(part 1 of 2)
# Autodesk Inventor assembly: gasienica_zlozenie
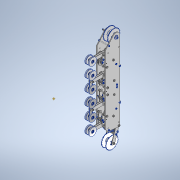
[picture p0: Inventor's stored thumbnail of the model, 180x180]
Saved by Autodesk Inventor 2020.3 (Build 243373000, 373)
## iProperties
Created: 2021-10-24
Part Number: gasienica_zlozenie
Document SubType Name: Assembly
Designer: patry
Author: patry
## Documents named in this file (46)
- C:\Users\patry\Desktop\Semestr 7\Inzynierka\Projekt inventor\Ariadna_inzynierka\Workspaces\Obszar roboczy\Obszar roboczy\Naped\Zawieszenie_v3\gasienica_zlozenie.iam
- C:\Users\patry\Desktop\Semestr 7\Inzynierka\Projekt inventor\Ariadna_inzynierka\Workspaces\Obszar roboczy\Obszar roboczy\Naped\Kola\kolo_przednie.iam
- C:\Users\patry\Desktop\Semestr 7\Inzynierka\Projekt inventor\Ariadna_inzynierka\Workspaces\Obszar roboczy\Obszar roboczy\Naped\Sruby\M5x65.ipt
- C:\Users\patry\Desktop\Semestr 7\Inzynierka\Projekt inventor\Ariadna_inzynierka\Workspaces\Obszar roboczy\Obszar roboczy\Naped\Sruby\M5_nut_5mm.ipt
- C:\Users\patry\Desktop\Semestr 7\Inzynierka\Projekt inventor\Ariadna_inzynierka\Workspaces\Obszar roboczy\Obszar roboczy\Naped\Sruby\dystans_miedzy_plytami.ipt
- C:\Users\patry\Desktop\Semestr 7\Inzynierka\Projekt inventor\Ariadna_inzynierka\Workspaces\Obszar roboczy\Obszar roboczy\Naped\Zawieszenie_v3\tuleja_TUF106040.ipt
- C:\Users\patry\Desktop\Semestr 7\Inzynierka\Projekt inventor\Ariadna_inzynierka\Workspaces\Obszar roboczy\Obszar roboczy\Naped\Sruby\M6_nut_5mm.ipt
- C:\Users\patry\Desktop\Semestr 7\Inzynierka\Projekt inventor\Ariadna_inzynierka\Workspaces\Obszar roboczy\Obszar roboczy\Naped\Amortyzator\Korpus.ipt
- C:\Users\patry\Desktop\Semestr 7\Inzynierka\Projekt inventor\Ariadna_inzynierka\Workspaces\Obszar roboczy\Obszar roboczy\Naped\Amortyzator\Tlok.ipt
- C:\Users\patry\Desktop\Semestr 7\Inzynierka\Projekt inventor\Ariadna_inzynierka\Workspaces\Obszar roboczy\Obszar roboczy\Naped\Amortyzator\Nakretka.ipt
- C:\Users\patry\Desktop\Semestr 7\Inzynierka\Projekt inventor\Ariadna_inzynierka\Workspaces\Obszar roboczy\Obszar roboczy\Naped\Sruby\M8_nut_6.5mm_MIR1.ipt
- C:\Users\patry\Desktop\Semestr 7\Inzynierka\Projekt inventor\Ariadna_inzynierka\Workspaces\Obszar roboczy\Obszar roboczy\Naped\Sruby\M8x80_threaded_MIR1.ipt
- C:\Users\patry\Desktop\Semestr 7\Inzynierka\Projekt inventor\Ariadna_inzynierka\Workspaces\Obszar roboczy\Obszar roboczy\Naped\Sruby\M8_pad_MIR1.ipt
- C:\Users\patry\Desktop\Semestr 7\Inzynierka\Projekt inventor\Ariadna_inzynierka\Workspaces\Obszar roboczy\Obszar roboczy\Naped\Lozyska\608ZZ-8mm\bearings-608zz-80018-1.snapshot.1\608zz_MIR1.ipt
- C:\Users\patry\Desktop\Semestr 7\Inzynierka\Projekt inventor\Ariadna_inzynierka\Workspaces\Obszar roboczy\Obszar roboczy\Naped\Kola\kolo_napedowe.iam
- C:\Users\patry\Desktop\Semestr 7\Inzynierka\Projekt inventor\Ariadna_inzynierka\Workspaces\Obszar roboczy\Obszar roboczy\Naped\Sruby\M5_70_shaft.ipt
- C:\Users\patry\Desktop\Semestr 7\Inzynierka\Projekt inventor\Ariadna_inzynierka\Workspaces\Obszar roboczy\Obszar roboczy\Naped\Sruby\M3_16_shaft.ipt
- C:\Users\patry\Desktop\Semestr 7\Inzynierka\Projekt inventor\Ariadna_inzynierka\Workspaces\Obszar roboczy\Obszar roboczy\Naped\Sruby\M3_nut_2,5mm.ipt
- C:\Users\patry\Desktop\Semestr 7\Inzynierka\Projekt inventor\Ariadna_inzynierka\Workspaces\Obszar roboczy\Obszar roboczy\Naped\Zawieszenie_v3\wspornik_amortyzatora.ipt
- C:\Users\patry\Desktop\Semestr 7\Inzynierka\Projekt inventor\Ariadna_inzynierka\Workspaces\Obszar roboczy\Obszar roboczy\Naped\Sruby\M6_70_shaft.ipt
- C:\Users\patry\Desktop\Semestr 7\Inzynierka\Projekt inventor\Ariadna_inzynierka\Workspaces\Obszar roboczy\Obszar roboczy\Naped\Sruby\tuleja_M5_M9_20.ipt
- C:\Users\patry\Desktop\Semestr 7\Inzynierka\Projekt inventor\Ariadna_inzynierka\Workspaces\Obszar roboczy\Obszar roboczy\Naped\Sruby\tuleja_M5_M9_25.ipt
- C:\Users\patry\Desktop\Semestr 7\Inzynierka\Projekt inventor\Ariadna_inzynierka\Workspaces\Obszar roboczy\Obszar roboczy\Naped\Kola\holder_wheel_pair.iam
- C:\Users\patry\Desktop\Semestr 7\Inzynierka\Projekt inventor\Ariadna_inzynierka\Workspaces\Obszar roboczy\Obszar roboczy\Naped\Zawieszenie_v3\ramie_napinacza.ipt
- C:\Users\patry\Desktop\Semestr 7\Inzynierka\Projekt inventor\Ariadna_inzynierka\Workspaces\Obszar roboczy\Obszar roboczy\Naped\Sruby\M5_60_shaft.ipt
- C:\Users\patry\Desktop\Semestr 7\Inzynierka\Projekt inventor\Ariadna_inzynierka\Workspaces\Obszar roboczy\Obszar roboczy\Naped\Sruby\tuleja_M5_M9_13.ipt
- C:\Users\patry\Desktop\Semestr 7\Inzynierka\Projekt inventor\Ariadna_inzynierka\Workspaces\Obszar roboczy\Obszar roboczy\Naped\Sruby\tuleja_M5_M9_18.ipt
- C:\Users\patry\Desktop\Semestr 7\Inzynierka\Projekt inventor\Ariadna_inzynierka\Workspaces\Obszar roboczy\Obszar roboczy\Naped\Sruby\tuleja_M6_M10_8.ipt
- C:\Users\patry\Desktop\Semestr 7\Inzynierka\Projekt inventor\Ariadna_inzynierka\Workspaces\Obszar roboczy\Obszar roboczy\Naped\Zawieszenie_v3\plyta_boczna.ipt
- C:\Users\patry\Desktop\Semestr 7\Inzynierka\Projekt inventor\Ariadna_inzynierka\Workspaces\Obszar roboczy\Obszar roboczy\Naped\Zawieszenie_v3\ramie_1_wahacza.ipt
- C:\Users\patry\Desktop\Semestr 7\Inzynierka\Projekt inventor\Ariadna_inzynierka\Workspaces\Obszar roboczy\Obszar roboczy\Naped\Zawieszenie_v3\ramie_2_wahacza.ipt
- C:\Users\patry\Desktop\Semestr 7\Inzynierka\Projekt inventor\Ariadna_inzynierka\Workspaces\Obszar roboczy\Obszar roboczy\Naped\Sruby\M6_40_shaft.ipt
- C:\Users\patry\Desktop\Semestr 7\Inzynierka\Projekt inventor\Ariadna_inzynierka\Workspaces\Obszar roboczy\Obszar roboczy\Naped\Sruby\tuleja_M6_M10_7.ipt
- C:\Users\patry\Desktop\Semestr 7\Inzynierka\Projekt inventor\Ariadna_inzynierka\Workspaces\Obszar roboczy\Obszar roboczy\Naped\Sruby\M6_1,25_pad.ipt
- C:\Users\patry\Desktop\Semestr 7\Inzynierka\Projekt inventor\Ariadna_inzynierka\Workspaces\Obszar roboczy\Obszar roboczy\Naped\Sruby\M5_40_shaft.ipt
- M5_shaft.ipt
- C:\Users\patry\Desktop\Semestr 7\Inzynierka\Projekt inventor\Ariadna_inzynierka\Workspaces\Obszar roboczy\Obszar roboczy\Naped\Sruby\tuleja_M5_M9_4,5.ipt
- C:\Users\patry\Desktop\Semestr 7\Inzynierka\Projekt inventor\Ariadna_inzynierka\Workspaces\Obszar roboczy\Obszar roboczy\Naped\Zawieszenie_v3\glowny_wahacz_zewn.ipt
- C:\Users\patry\Desktop\Semestr 7\Inzynierka\Projekt inventor\Ariadna_inzynierka\Workspaces\Obszar roboczy\Obszar roboczy\Naped\Zawieszenie_v3\independent_wheel_pair.iam
- C:\Users\patry\Desktop\Semestr 7\Inzynierka\Projekt inventor\Ariadna_inzynierka\Workspaces\Obszar roboczy\Obszar roboczy\Naped\Sruby\tuleja_M6_M10_6.ipt
- C:\Users\patry\Desktop\Semestr 7\Inzynierka\Projekt inventor\Ariadna_inzynierka\Workspaces\Obszar roboczy\Obszar roboczy\Naped\Sruby\tuleja_M5_M9_17.5.ipt
- C:\Users\patry\Desktop\Semestr 7\Inzynierka\Projekt inventor\Ariadna_inzynierka\Workspaces\Obszar roboczy\Obszar roboczy\Naped\Zawieszenie_v3\komplet_kol_V4.iam
- C:\Users\patry\Desktop\Semestr 7\Inzynierka\Projekt inventor\Ariadna_inzynierka\Workspaces\Obszar roboczy\Obszar roboczy\Naped\Sruby\M6_25_shaft.ipt
- C:\Users\patry\Desktop\Semestr 7\Inzynierka\Projekt inventor\Ariadna_inzynierka\Workspaces\Obszar roboczy\Obszar roboczy\Naped\Kola\single_wheel_dummie.iam
- C:\Users\patry\Desktop\Semestr 7\Inzynierka\Projekt inventor\Ariadna_inzynierka\Workspaces\Obszar roboczy\Obszar roboczy\Naped\Sruby\tuleja_M5_M10_15.ipt
- C:\Users\patry\Desktop\Semestr 7\Inzynierka\Projekt inventor\Ariadna_inzynierka\Workspaces\Obszar roboczy\Obszar roboczy\Naped\Sruby\tuleja_M6_M10_7,5.ipt
## Components (345 placed, 44 different names)
1. M5x65:3
2. M5_nut_5mm:3
3. dystans_miedzy_plytami:3
4. M8_nut_6.5mm_MIR1:1
5. M8x80_threaded_MIR1:1
6. M8_nut_6.5mm_MIR1:2
7. M8_nut_6.5mm_MIR1:3
8. M8_pad_MIR1:1
9. M8_pad_MIR1:2
10. M8_pad_MIR1:3
11. M8_pad_MIR1:4
12. 608zz_MIR1:1
13. 608zz_MIR1:2 — Zestawiające:1077, Równoległe:74
14. kolo_napedowe:1 [sub-assembly]
15. kolo_przednie:1 [sub-assembly]
16. ramie_napinacza:1 — Zestawiające:1807
17. Korpus:6 — Walcowe:6
18. Tlok:6 — Walcowe:6
19. Nakretka:6
20. M5_nut_5mm:34
21. M5_70_shaft:6 — Zestawiające:1080
22. M5_nut_5mm:35
23. M3_16_shaft:6
24. M3_nut_2,5mm:11
25. M3_nut_2,5mm:12
26. wspornik_amortyzatora:11 — Zestawiające:1086, Zestawiające:1087
27. wspornik_amortyzatora:12
28. M5_nut_5mm:36
29. M5_nut_5mm:37
30. M5_nut_5mm:38
31. M5_nut_5mm:39
32. tuleja_M5_M9_20:6
33. tuleja_M5_M9_25:6
34. ramie_napinacza:2 — Zestawiające:1804
35. M5_60_shaft:1 — Zestawiające:1086
36. M5_60_shaft:2 — Zestawiające:1087, Zestawiające:1796, Zestawiające:1797
37. tuleja_TUF106040:41 — Zestawiające:1085
38. tuleja_TUF106040:42
39. M6_70_shaft:11 — Zestawiające:1079, Zestawiające:1802, Zestawiające:1803, Zestawiające:1806
40. M6_nut_5mm:49
41. M6_nut_5mm:50
42. tuleja_M5_M9_13:1 — Zestawiające:1796
43. tuleja_M5_M9_18:1 — Zestawiające:1797
44. M6_70_shaft:12
45. M6_nut_5mm:51
46. M6_nut_5mm:52
47. tuleja_M6_M10_8:1
48. tuleja_M6_M10_8:2
49. holder_wheel_pair:4 [sub-assembly] — Zestawiające:1082, Zestawiające:1083
50. holder_wheel_pair:5 [sub-assembly] — Zestawiające:1081, Zestawiające:1084
51. plyta_boczna:1 — Zestawiające:1075, Zestawiające:1076, Zestawiające:1077, Zestawiające:1078, Równoległe:74, Kątowe:22, Zestawiające:1079, Zestawiające:1080, Zestawiające:1081, Zestawiające:1082, Zestawiające:1083, Zestawiające:1084, Zestawiające:1085, Zestawiające:1632, Zestawiające:1633, Kątowe:49
52. plyta_boczna:2 — Zestawiające:1075, Zestawiające:1076, Zestawiające:1078, Zestawiające:1222, Zestawiające:1224, Zestawiające:1225, Zestawiające:1226, Zestawiające:1636, Zestawiające:1637, Zestawiające:1638, Zestawiające:1639, Zestawiające:1640, Zestawiające:1641, Zestawiające:1777, Zestawiające:1778, Zestawiające:1779, Zestawiające:1780
53. ramie_1_wahacza:1
54. ramie_2_wahacza:1
55. tuleja_TUF106040:43
56. tuleja_TUF106040:44
57. tuleja_TUF106040:45
58. tuleja_TUF106040:46
59. tuleja_TUF106040:47
60. tuleja_TUF106040:48
61. ramie_2_wahacza:2
62. tuleja_TUF106040:49
63. tuleja_TUF106040:50
64. M6_nut_5mm:53
65. Korpus:7
66. Tlok:7
67. Nakretka:7
68. M5_nut_5mm:40
69. M5_70_shaft:7
70. ramie_1_wahacza:2 — Kątowe:27
71. M5_nut_5mm:41
72. M3_16_shaft:7
73. M3_nut_2,5mm:13
74. M3_nut_2,5mm:14
75. wspornik_amortyzatora:13
76. wspornik_amortyzatora:14
77. M6_40_shaft:1
78. M6_40_shaft:2
79. M6_nut_5mm:54
80. M6_nut_5mm:55
81. M6_nut_5mm:56
82. tuleja_M6_M10_7:1
83. tuleja_M6_M10_7:2
84. M6_1,25_pad:1
85. M6_1,25_pad:2
86. M6_1,25_pad:3
87. M6_1,25_pad:4
88. M6_1,25_pad:5
89. M6_1,25_pad:6
90. M6_1,25_pad:7
91. M6_1,25_pad:8
92. M6_70_shaft:13 — Zestawiające:1225
93. M6_70_shaft:14 — Zestawiające:1222
94. M6_nut_5mm:57
95. M6_nut_5mm:58 — Zestawiające:1224
96. M6_nut_5mm:59
97. M6_nut_5mm:60
98. M5_shaft:1
99. M5_shaft:2
100. M5_nut_5mm:42
101. M5_nut_5mm:43
102. M5_nut_5mm:44
103. M5_nut_5mm:45
104. tuleja_M5_M9_4,5:1
105. tuleja_M5_M9_4,5:2
106. tuleja_M5_M9_4,5:3
107. tuleja_M5_M9_4,5:4
108. glowny_wahacz_zewn:1 — Zestawiające:1223, Kątowe:27
109. glowny_wahacz_zewn:2
110. independent_wheel_pair:1 [sub-assembly]
111. tuleja_M6_M10_7:3 — Zestawiające:1223
112. tuleja_M6_M10_6:1
113. M6_nut_5mm:61
114. M6_nut_5mm:62
115. M6_nut_5mm:63
116. M6_nut_5mm:64
117. tuleja_M6_M10_6:2
118. tuleja_M6_M10_6:3
119. tuleja_M6_M10_6:4
120. M5_nut_5mm:46
121. M5_nut_5mm:47
122. tuleja_M5_M9_17.5:1
123. tuleja_M5_M9_17.5:2 — Zestawiające:1226
124. ramie_1_wahacza:3
125. ramie_2_wahacza:3
126. tuleja_TUF106040:51
127. tuleja_TUF106040:52
128. tuleja_TUF106040:53
129. tuleja_TUF106040:54
130. tuleja_TUF106040:55
131. tuleja_TUF106040:56
132. ramie_2_wahacza:4
133. tuleja_TUF106040:57
134. tuleja_TUF106040:58
135. M6_nut_5mm:65
136. Korpus:8
137. Tlok:8
138. Nakretka:8
139. M5_nut_5mm:48
140. M5_70_shaft:8
141. ramie_1_wahacza:4 — Kątowe:40
142. M5_nut_5mm:49
143. M3_16_shaft:8
144. M3_nut_2,5mm:15
145. M3_nut_2,5mm:16
146. wspornik_amortyzatora:15
147. wspornik_amortyzatora:16
148. M6_40_shaft:3
149. M6_40_shaft:4
150. M6_nut_5mm:66
151. M6_nut_5mm:67
152. M6_nut_5mm:68
153. tuleja_M6_M10_7:4
154. tuleja_M6_M10_7:5
155. M6_1,25_pad:9
156. M6_1,25_pad:10
157. M6_1,25_pad:11
158. M6_1,25_pad:12
159. M6_1,25_pad:13
160. M6_1,25_pad:14
161. M6_1,25_pad:15
162. M6_1,25_pad:16
163. M6_70_shaft:15 — Zestawiające:1636
164. M6_70_shaft:16 — Zestawiające:1632
165. M6_nut_5mm:69
166. M6_nut_5mm:70
167. M6_nut_5mm:71
168. M6_nut_5mm:72
169. M5_shaft:3
170. M5_shaft:4
171. M5_nut_5mm:50
172. M5_nut_5mm:51
173. M5_nut_5mm:52
174. M5_nut_5mm:53
175. tuleja_M5_M9_4,5:5
176. tuleja_M5_M9_4,5:6
177. tuleja_M5_M9_4,5:7
178. tuleja_M5_M9_4,5:8
179. glowny_wahacz_zewn:3 — Kątowe:40, Zestawiające:1793, Zestawiające:1794, Zestawiające:1795
180. glowny_wahacz_zewn:4 — Zestawiające:1793
181. tuleja_M6_M10_6:5
182. M6_nut_5mm:73
183. M6_nut_5mm:74
184. M6_nut_5mm:75 — Zestawiające:1633
185. M6_nut_5mm:76
186. tuleja_M6_M10_6:6
187. tuleja_M6_M10_6:7
188. tuleja_M6_M10_6:8
189. M5_nut_5mm:54
190. M5_nut_5mm:55
191. tuleja_M5_M9_17.5:3 — Zestawiające:1637
192. tuleja_M5_M9_17.5:4
193. ramie_1_wahacza:7 — Kątowe:41
194. ramie_2_wahacza:7
195. tuleja_TUF106040:67
196. tuleja_TUF106040:68
197. tuleja_TUF106040:69
198. tuleja_TUF106040:70
199. tuleja_TUF106040:71
200. tuleja_TUF106040:72
201. ramie_2_wahacza:8
202. tuleja_TUF106040:73
203. tuleja_TUF106040:74
204. M6_nut_5mm:89
205. Korpus:10
206. Tlok:10
207. Nakretka:10
208. M5_nut_5mm:64
209. M5_70_shaft:10
210. ramie_1_wahacza:8
211. M5_nut_5mm:65 — Zestawiające:1638
212. M3_16_shaft:10
213. M3_nut_2,5mm:19
214. M3_nut_2,5mm:20
215. wspornik_amortyzatora:19
216. wspornik_amortyzatora:20
217. M6_40_shaft:7
218. M6_40_shaft:8
219. M6_nut_5mm:90
220. M6_nut_5mm:91
221. M6_nut_5mm:92
222. tuleja_M6_M10_7:10
223. tuleja_M6_M10_7:11
224. M6_1,25_pad:25
225. M6_1,25_pad:26
226. M6_1,25_pad:27
227. M6_1,25_pad:28
228. M6_1,25_pad:29
229. M6_1,25_pad:30
230. M6_1,25_pad:31
231. M6_1,25_pad:32
232. M6_70_shaft:19 — Zestawiające:1640
233. M6_70_shaft:20 — Zestawiające:1639
234. M6_nut_5mm:93
235. M6_nut_5mm:94
236. M6_nut_5mm:95
237. M6_nut_5mm:96
238. M5_shaft:7
239. M5_shaft:8
240. M5_nut_5mm:66
241. M5_nut_5mm:67
242. M5_nut_5mm:68
243. M5_nut_5mm:69
244. tuleja_M5_M9_4,5:13
245. tuleja_M5_M9_4,5:14
246. tuleja_M5_M9_4,5:15
247. tuleja_M5_M9_4,5:16
248. glowny_wahacz_zewn:7 — Zestawiające:1784
249. glowny_wahacz_zewn:8 — Kątowe:41, Zestawiające:1781, Zestawiające:1782, Zestawiające:1789
250. tuleja_M6_M10_6:13
251. M6_nut_5mm:97
252. M6_nut_5mm:98
253. M6_nut_5mm:99
254. M6_nut_5mm:100
255. tuleja_M6_M10_6:14
256. tuleja_M6_M10_6:15
257. tuleja_M6_M10_6:16
258. M5_nut_5mm:70
259. M5_nut_5mm:71
260. tuleja_M5_M9_17.5:7 — Zestawiające:1641
261. tuleja_M5_M9_17.5:8
262. ramie_1_wahacza:9 — Kątowe:47
263. ramie_2_wahacza:9
264. tuleja_TUF106040:75
265. tuleja_TUF106040:76
266. tuleja_TUF106040:77
267. tuleja_TUF106040:78
268. tuleja_TUF106040:79
269. tuleja_TUF106040:80
270. ramie_2_wahacza:10
271. tuleja_TUF106040:81
272. tuleja_TUF106040:82
273. M6_nut_5mm:101
274. Korpus:11
275. Tlok:11
276. Nakretka:11
277. M5_nut_5mm:72
278. M5_70_shaft:11
279. ramie_1_wahacza:10
280. M5_nut_5mm:73
281. M3_16_shaft:11
282. M3_nut_2,5mm:21
283. M3_nut_2,5mm:22
284. wspornik_amortyzatora:21
285. wspornik_amortyzatora:22
286. M6_40_shaft:9
287. M6_40_shaft:10
288. M6_nut_5mm:102
289. M6_nut_5mm:103
290. M6_nut_5mm:104
291. tuleja_M6_M10_7:13
292. tuleja_M6_M10_7:14
293. M6_1,25_pad:33
294. M6_1,25_pad:34
295. M6_1,25_pad:35
296. M6_1,25_pad:36
297. M6_1,25_pad:37
298. M6_1,25_pad:38
299. M6_1,25_pad:39
300. M6_1,25_pad:40
301. M6_70_shaft:21 — Zestawiające:1779
302. M6_70_shaft:22 — Zestawiające:1778
303. M6_nut_5mm:105
304. M6_nut_5mm:106
305. M6_nut_5mm:107 — Zestawiające:1777
306. M6_nut_5mm:108
307. M5_shaft:9
308. M5_shaft:10
309. M5_nut_5mm:74
310. M5_nut_5mm:75
311. M5_nut_5mm:76
312. M5_nut_5mm:77
313. tuleja_M5_M9_4,5:17
314. tuleja_M5_M9_4,5:18
315. tuleja_M5_M9_4,5:19
316. tuleja_M5_M9_4,5:20
317. glowny_wahacz_zewn:9
318. glowny_wahacz_zewn:10 — Kątowe:47
319. independent_wheel_pair:5 [sub-assembly]
320. tuleja_M6_M10_7:15
321. tuleja_M6_M10_6:17
322. M6_nut_5mm:109
323. M6_nut_5mm:110
324. M6_nut_5mm:111
325. M6_nut_5mm:112
326. tuleja_M6_M10_6:18
327. tuleja_M6_M10_6:19
328. tuleja_M6_M10_6:20
329. M5_nut_5mm:78
330. M5_nut_5mm:79
331. tuleja_M5_M9_17.5:9
332. tuleja_M5_M9_17.5:10 — Zestawiające:1780
333. komplet_kol_V4:1 [sub-assembly] — Zestawiające:1781, Zestawiające:1782, Zestawiające:1784, Zestawiające:1788, Kątowe:48
334. M6_nut_5mm:115 — Zestawiające:1789
335. M6_25_shaft:2 — Zestawiające:1788
336. M6_nut_5mm:116
337. komplet_kol_V4:2 [sub-assembly] — Zestawiające:1795, Kątowe:48, Kątowe:49
338. M6_nut_5mm:117
339. M6_25_shaft:3 — Zestawiające:1794
340. M6_nut_5mm:118
341. single_wheel_dummie:1 [sub-assembly] — Zestawiające:1799
342. single_wheel_dummie:2 [sub-assembly] — Zestawiające:1800, Zestawiające:1801, Zestawiające:1802, Zestawiające:1805
343. tuleja_M5_M10_15:1 — Zestawiające:1799, Zestawiające:1800, Zestawiające:1801
344. tuleja_M6_M10_7,5:1 — Zestawiające:1803, Zestawiające:1804, Zestawiające:1805
345. tuleja_M6_M10_7,5:2 — Zestawiające:1806, Zestawiające:1807
## Relationships (742: Mate 664, Flush 49, Angle 24, CylindricalJoint 5)
- [Mate]: M5x65:3 ↔ M5_nut_5mm:3
- [Flush]: M5x65:3 ↔ M5_nut_5mm:3
- [Mate]: M5x65:3 ↔ dystans_miedzy_plytami:3
- [Mate] (5 mm): M5x65:3 ↔ dystans_miedzy_plytami:3
- [Mate]: M8_nut_6.5mm_MIR1:1 ↔ M8x80_threaded_MIR1:1
- [Mate]: M8x80_threaded_MIR1:1 ↔ M8_nut_6.5mm_MIR1:2
- [Mate]: M8x80_threaded_MIR1:1 ↔ M8_nut_6.5mm_MIR1:3
- [Mate]: M8_nut_6.5mm_MIR1:1 ↔ M8_pad_MIR1:1
- [Mate] (7 mm): M8x80_threaded_MIR1:1 ↔ M8_pad_MIR1:1
- [Mate]: M8x80_threaded_MIR1:1 ↔ M8_pad_MIR1:1
- [Mate]: M8_nut_6.5mm_MIR1:1 ↔ M8_pad_MIR1:2
- [Mate]: M8x80_threaded_MIR1:1 ↔ M8_pad_MIR1:2
- [Mate] (7 mm): M8_nut_6.5mm_MIR1:2 ↔ M8_pad_MIR1:3
- [Mate]: M8_nut_6.5mm_MIR1:3 ↔ M8_pad_MIR1:3
- [Mate]: M8x80_threaded_MIR1:1 ↔ M8_pad_MIR1:3
- [Mate]: M8_nut_6.5mm_MIR1:3 ↔ M8_pad_MIR1:4
- [Mate] (31 mm): M8_pad_MIR1:2 ↔ M8_pad_MIR1:4
- [Mate]: M8x80_threaded_MIR1:1 ↔ M8_pad_MIR1:4
- [Mate]: M8x80_threaded_MIR1:1 ↔ 608zz_MIR1:1
- [Mate]: M8_nut_6.5mm_MIR1:2 ↔ 608zz_MIR1:1
- [Mate]: M8x80_threaded_MIR1:1 ↔ 608zz_MIR1:2
- [Mate]: M8x80_threaded_MIR1:1 ↔ 608zz_MIR1:2
- [Mate]: M8x80_threaded_MIR1:1 ↔ kolo_napedowe:1
- [Mate]: M8_pad_MIR1:2 ↔ kolo_napedowe:1
- [Mate]: Korpus:6 ↔ Tlok:6
- [Angle] (0 deg): Korpus:6 ↔ Tlok:6
- [Mate]: Korpus:6 ↔ Nakretka:6
- [Mate] (5 mm): Korpus:6 ↔ Nakretka:6
- Walcowe:6 [CylindricalJoint]: Korpus:6 ↔ Tlok:6
- [Mate]: Korpus:6 ↔ M5_70_shaft:6
- [Flush] (-30 mm): Korpus:6 ↔ M5_70_shaft:6
- [Mate]: M5_nut_5mm:34 ↔ M5_70_shaft:6
- [Mate]: M5_70_shaft:6 ↔ M5_nut_5mm:35
- [Mate] (60 mm): M5_nut_5mm:34 ↔ M5_nut_5mm:35
- [Mate] (30 mm): Korpus:6 ↔ M5_nut_5mm:34
- [Mate]: wspornik_amortyzatora:11 ↔ wspornik_amortyzatora:12
- [Mate]: wspornik_amortyzatora:11 ↔ wspornik_amortyzatora:12
- [Mate] (5 mm): wspornik_amortyzatora:11 ↔ wspornik_amortyzatora:12
- [Mate]: M3_16_shaft:6 ↔ wspornik_amortyzatora:12
- [Flush] (-2.5 mm): M3_16_shaft:6 ↔ wspornik_amortyzatora:11
- [Mate]: M3_16_shaft:6 ↔ M3_nut_2,5mm:11
- [Mate]: M3_nut_2,5mm:11 ↔ wspornik_amortyzatora:11
- [Mate]: M3_16_shaft:6 ↔ M3_nut_2,5mm:12
- [Mate]: M3_nut_2,5mm:12 ↔ wspornik_amortyzatora:12
- [Mate]: Tlok:6 ↔ M3_16_shaft:6
- [Mate]: Tlok:6 ↔ wspornik_amortyzatora:12
- [Mate]: M5_70_shaft:6 ↔ tuleja_M5_M9_20:6
- [Mate]: Korpus:6 ↔ tuleja_M5_M9_20:6
- [Mate]: M5_70_shaft:6 ↔ tuleja_M5_M9_25:6
- [Mate]: Korpus:6 ↔ tuleja_M5_M9_25:6
- [Mate]: M6_70_shaft:11 ↔ M6_nut_5mm:49
- [Mate]: M6_70_shaft:11 ↔ M6_nut_5mm:50
- [Mate] (60 mm): M6_nut_5mm:49 ↔ M6_nut_5mm:50
- [Mate]: tuleja_TUF106040:41 ↔ M6_70_shaft:11
- [Mate]: ramie_napinacza:1 ↔ ramie_napinacza:2
- [Mate]: ramie_napinacza:1 ↔ ramie_napinacza:2
- [Mate] (42 mm): ramie_napinacza:1 ↔ ramie_napinacza:2
- [Mate]: ramie_napinacza:1 ↔ tuleja_TUF106040:41
- [Mate]: ramie_napinacza:1 ↔ tuleja_TUF106040:41
- [Mate]: ramie_napinacza:2 ↔ tuleja_TUF106040:42
- [Mate]: ramie_napinacza:2 ↔ tuleja_TUF106040:42
- [Mate] (5 mm): tuleja_TUF106040:41 ↔ M6_nut_5mm:49
- [Flush] (-11 mm): ramie_napinacza:2 ↔ M6_70_shaft:11
- [Mate] (5.5 mm): kolo_przednie:1 ↔ ramie_napinacza:1
- [Mate]: kolo_przednie:1 ↔ ramie_napinacza:1
- [Mate]: ramie_napinacza:1 ↔ M5_60_shaft:1
- [Flush] (6 mm): ramie_napinacza:1 ↔ M5_60_shaft:1
- [Mate]: ramie_napinacza:1 ↔ M5_60_shaft:2
- [Flush] (6 mm): ramie_napinacza:1 ↔ M5_60_shaft:2
- [Mate]: M5_nut_5mm:37 ↔ M5_60_shaft:1
- [Mate]: ramie_napinacza:1 ↔ M5_nut_5mm:37
- [Mate]: M5_nut_5mm:38 ↔ M5_60_shaft:1
- [Mate]: M5_nut_5mm:38 ↔ ramie_napinacza:2
- [Mate]: M5_nut_5mm:39 ↔ M5_60_shaft:2
- [Mate]: M5_nut_5mm:39 ↔ ramie_napinacza:2
- [Mate]: M5_nut_5mm:36 ↔ M5_60_shaft:2
- [Mate]: ramie_napinacza:1 ↔ M5_nut_5mm:36
- [Flush]: M5_nut_5mm:34 ↔ M6_nut_5mm:50
- [Mate]: wspornik_amortyzatora:12 ↔ tuleja_M5_M9_18:1
- [Mate]: ramie_napinacza:1 ↔ tuleja_M5_M9_13:1
- [Mate]: ramie_napinacza:1 ↔ M6_70_shaft:12
- [Flush] (-11 mm): ramie_napinacza:1 ↔ M6_70_shaft:12
- [Mate]: M6_70_shaft:12 ↔ M6_nut_5mm:51
- [Mate]: ramie_napinacza:1 ↔ M6_nut_5mm:51
- [Mate]: M6_70_shaft:12 ↔ M6_nut_5mm:52
- [Mate]: ramie_napinacza:2 ↔ M6_nut_5mm:52
- [Mate]: M6_70_shaft:12 ↔ tuleja_M6_M10_8:1
- [Mate]: ramie_napinacza:1 ↔ tuleja_M6_M10_8:1
- [Mate]: M6_70_shaft:12 ↔ tuleja_M6_M10_8:2
- [Mate]: ramie_napinacza:2 ↔ tuleja_M6_M10_8:2
- Zestawiające:1075 [Mate]: plyta_boczna:1 ↔ plyta_boczna:2
- Zestawiające:1076 [Mate]: plyta_boczna:1 ↔ plyta_boczna:2
- Zestawiające:1077 [Mate]: 608zz_MIR1:2 ↔ plyta_boczna:1
- Zestawiające:1078 [Mate] (50 mm): plyta_boczna:1 ↔ plyta_boczna:2
- Równoległe:74 [Flush] (-1 mm): 608zz_MIR1:2 ↔ plyta_boczna:1
- Kątowe:22 [Angle] (180 deg): plyta_boczna:1
- Zestawiające:1079 [Mate]: M6_70_shaft:11 ↔ plyta_boczna:1
- Zestawiające:1080 [Mate]: M5_70_shaft:6 ↔ plyta_boczna:1
- Zestawiające:1081 [Mate]: holder_wheel_pair:5 ↔ plyta_boczna:1
- Zestawiające:1082 [Mate]: holder_wheel_pair:4 ↔ plyta_boczna:1
- Zestawiające:1083 [Mate]: holder_wheel_pair:4 ↔ plyta_boczna:1
- Zestawiające:1084 [Mate]: holder_wheel_pair:5 ↔ plyta_boczna:1
- Zestawiające:1085 [Mate]: tuleja_TUF106040:41 ↔ plyta_boczna:1
- Zestawiające:1086 [Mate]: wspornik_amortyzatora:11 ↔ M5_60_shaft:1
- Zestawiające:1087 [Mate]: wspornik_amortyzatora:11 ↔ M5_60_shaft:2
- [Mate]: ramie_2_wahacza:1 ↔ tuleja_TUF106040:43
- [Mate]: ramie_2_wahacza:1 ↔ tuleja_TUF106040:43
- [Angle] (0 deg): ramie_2_wahacza:1 ↔ tuleja_TUF106040:43
- [Mate]: ramie_1_wahacza:1 ↔ tuleja_TUF106040:46
- [Mate]: ramie_1_wahacza:1 ↔ tuleja_TUF106040:46
- [Angle] (0 deg): ramie_1_wahacza:1 ↔ tuleja_TUF106040:46
- [Mate]: ramie_2_wahacza:2 ↔ tuleja_TUF106040:49
- [Mate]: ramie_2_wahacza:2 ↔ tuleja_TUF106040:49
- [Angle] (0 deg): ramie_2_wahacza:2 ↔ tuleja_TUF106040:49
- [Mate]: Korpus:7 ↔ Tlok:7
- [Angle] (0 deg): Korpus:7 ↔ Tlok:7
- [Mate]: Korpus:7 ↔ Nakretka:7
- [Mate] (5 mm): Korpus:7 ↔ Nakretka:7
- [CylindricalJoint]: Korpus:7 ↔ Tlok:7
- [Mate]: Korpus:7 ↔ M5_70_shaft:7
- [Flush] (-32.5 mm): Korpus:7 ↔ M5_70_shaft:7
- [Mate]: M5_nut_5mm:40 ↔ M5_70_shaft:7
- [Mate]: M5_70_shaft:7 ↔ M5_nut_5mm:41
- [Mate] (60 mm): M5_nut_5mm:40 ↔ M5_nut_5mm:41
- [Mate] (27.5 mm): Korpus:7 ↔ M5_nut_5mm:40
- [Mate]: tuleja_TUF106040:48 ↔ ramie_1_wahacza:2
- [Mate]: tuleja_TUF106040:47 ↔ ramie_1_wahacza:2
- [Mate]: tuleja_TUF106040:48 ↔ ramie_1_wahacza:2
- [Mate]: tuleja_TUF106040:43 ↔ tuleja_TUF106040:49
- [Mate]: wspornik_amortyzatora:13 ↔ wspornik_amortyzatora:14
- [Mate]: wspornik_amortyzatora:13 ↔ wspornik_amortyzatora:14
- [Mate] (5 mm): wspornik_amortyzatora:13 ↔ wspornik_amortyzatora:14
- [Mate]: M3_16_shaft:7 ↔ wspornik_amortyzatora:14
- [Flush] (-2.5 mm): M3_16_shaft:7 ↔ wspornik_amortyzatora:13
- [Mate]: M3_16_shaft:7 ↔ M3_nut_2,5mm:13
- [Mate]: M3_nut_2,5mm:13 ↔ wspornik_amortyzatora:13
- [Mate]: M3_16_shaft:7 ↔ M3_nut_2,5mm:14
- [Mate]: M3_nut_2,5mm:14 ↔ wspornik_amortyzatora:14
- [Mate]: Tlok:7 ↔ M3_16_shaft:7
- [Mate]: Tlok:7 ↔ wspornik_amortyzatora:14
- [Mate]: ramie_1_wahacza:1 ↔ wspornik_amortyzatora:13
- [Mate]: ramie_1_wahacza:1 ↔ wspornik_amortyzatora:13
- [Mate] (4.5 mm): ramie_1_wahacza:1 ↔ wspornik_amortyzatora:13
- [Mate]: tuleja_TUF106040:46 ↔ M6_40_shaft:1
- [Flush] (7 mm): ramie_1_wahacza:1 ↔ M6_40_shaft:1
- [Mate]: tuleja_TUF106040:49 ↔ M6_40_shaft:2
- [Flush] (7 mm): ramie_2_wahacza:2 ↔ M6_40_shaft:2
- [Mate]: M6_nut_5mm:53 ↔ M6_40_shaft:1
- [Mate]: ramie_1_wahacza:1 ↔ M6_nut_5mm:53
- [Mate]: M6_40_shaft:1 ↔ M6_nut_5mm:54
- [Mate]: ramie_1_wahacza:2 ↔ M6_nut_5mm:54
- [Mate]: M6_40_shaft:2 ↔ M6_nut_5mm:55
- [Mate]: ramie_2_wahacza:1 ↔ M6_nut_5mm:55
- [Mate]: M6_40_shaft:2 ↔ M6_nut_5mm:56
- [Mate]: ramie_2_wahacza:2 ↔ M6_nut_5mm:56
- [Mate]: M6_40_shaft:1 ↔ tuleja_M6_M10_7:1
- [Mate]: M6_40_shaft:2 ↔ tuleja_M6_M10_7:2
- [Mate]: M6_1,25_pad:1 ↔ M6_1,25_pad:2
- [Mate]: M6_1,25_pad:1 ↔ M6_1,25_pad:2
- [Mate]: M6_40_shaft:1 ↔ M6_1,25_pad:1
- [Mate]: M6_1,25_pad:3 ↔ M6_1,25_pad:4
- [Mate]: M6_1,25_pad:3 ↔ M6_1,25_pad:4
- [Mate]: M6_40_shaft:1 ↔ M6_1,25_pad:3
- [Mate]: tuleja_TUF106040:46 ↔ M6_1,25_pad:3
- [Mate]: M6_1,25_pad:5 ↔ M6_1,25_pad:6
- [Mate]: M6_1,25_pad:5 ↔ M6_1,25_pad:6
- [Mate]: M6_40_shaft:2 ↔ M6_1,25_pad:5
- [Mate]: M6_1,25_pad:7 ↔ M6_1,25_pad:8
- [Mate]: M6_1,25_pad:7 ↔ M6_1,25_pad:8
- [Mate]: M6_40_shaft:2 ↔ M6_1,25_pad:7
- [Mate]: tuleja_TUF106040:49 ↔ M6_1,25_pad:7
- [Mate]: M5_70_shaft:7 ↔ M6_70_shaft:13
- [Flush]: M5_70_shaft:7 ↔ M6_70_shaft:14
- [Mate]: M6_70_shaft:14 ↔ M6_nut_5mm:57
- [Mate]: M6_70_shaft:14 ↔ M6_nut_5mm:58
- [Mate] (60 mm): M6_nut_5mm:57 ↔ M6_nut_5mm:58
- [Flush]: M5_nut_5mm:40 ↔ M6_nut_5mm:58
- [Mate] (60 mm): M6_nut_5mm:59 ↔ M6_nut_5mm:60
- [Mate]: M6_nut_5mm:59 ↔ M6_nut_5mm:60
- [Mate]: M6_70_shaft:13 ↔ M6_nut_5mm:59
- [Flush]: M5_nut_5mm:40 ↔ M6_nut_5mm:60
- [Mate]: ramie_1_wahacza:1 ↔ M5_shaft:1
- [Flush] (7 mm): ramie_1_wahacza:1 ↔ M5_shaft:1
- [Mate]: ramie_1_wahacza:1 ↔ M5_shaft:2
- [Flush] (7 mm): ramie_1_wahacza:1 ↔ M5_shaft:2
- [Mate]: M5_shaft:2 ↔ M5_nut_5mm:42
- [Mate]: ramie_1_wahacza:1 ↔ M5_nut_5mm:42
- [Mate]: M5_shaft:1 ↔ M5_nut_5mm:43
- [Mate]: ramie_1_wahacza:1 ↔ M5_nut_5mm:43
- [Mate]: M5_shaft:1 ↔ M5_nut_5mm:44
- [Mate]: ramie_1_wahacza:2 ↔ M5_nut_5mm:44
- [Mate]: M5_shaft:2 ↔ M5_nut_5mm:45
- [Mate]: ramie_1_wahacza:2 ↔ M5_nut_5mm:45
- [Mate]: M5_shaft:1 ↔ tuleja_M5_M9_4,5:1
- [Mate]: ramie_1_wahacza:2 ↔ tuleja_M5_M9_4,5:1
- [Mate]: M5_shaft:1 ↔ tuleja_M5_M9_4,5:2
- [Mate]: ramie_1_wahacza:1 ↔ tuleja_M5_M9_4,5:2
- [Mate]: M5_shaft:2 ↔ tuleja_M5_M9_4,5:3
- [Mate]: ramie_1_wahacza:2 ↔ tuleja_M5_M9_4,5:3
- [Mate]: M5_shaft:2 ↔ tuleja_M5_M9_4,5:4
- [Mate]: ramie_1_wahacza:1 ↔ tuleja_M5_M9_4,5:4
- [Mate]: M6_40_shaft:2 ↔ glowny_wahacz_zewn:1
- [Mate]: tuleja_M6_M10_7:2 ↔ glowny_wahacz_zewn:1
- [Mate]: M6_40_shaft:1 ↔ glowny_wahacz_zewn:1
- [Mate]: M6_40_shaft:2 ↔ glowny_wahacz_zewn:2
- [Mate]: M6_40_shaft:1 ↔ glowny_wahacz_zewn:2
- [Mate]: tuleja_TUF106040:48 ↔ M6_40_shaft:1
- [Mate]: M6_1,25_pad:4 ↔ glowny_wahacz_zewn:2
- [Mate]: M6_1,25_pad:8 ↔ glowny_wahacz_zewn:2
- [Mate]: tuleja_M6_M10_7:1 ↔ glowny_wahacz_zewn:1
- [Mate]: M6_1,25_pad:1 ↔ glowny_wahacz_zewn:1
- [Mate]: tuleja_TUF106040:48 ↔ M6_1,25_pad:2
- [Mate]: M6_1,25_pad:5 ↔ glowny_wahacz_zewn:1
- [Mate]: tuleja_TUF106040:43 ↔ M6_1,25_pad:6
- [Mate]: tuleja_TUF106040:47 ↔ ramie_1_wahacza:2
- [Mate]: tuleja_TUF106040:45 ↔ M6_70_shaft:14
- [Mate]: ramie_1_wahacza:1 ↔ tuleja_TUF106040:45
- [Mate]: ramie_1_wahacza:1 ↔ tuleja_TUF106040:45
- [Mate]: tuleja_TUF106040:44 ↔ M6_70_shaft:13
- [Mate]: ramie_2_wahacza:1 ↔ tuleja_TUF106040:44
- [Mate]: ramie_2_wahacza:1 ↔ tuleja_TUF106040:44
- [Mate]: tuleja_TUF106040:50 ↔ M6_70_shaft:13
- [Mate]: ramie_2_wahacza:2 ↔ tuleja_TUF106040:50
- [Mate]: ramie_2_wahacza:2 ↔ tuleja_TUF106040:50
- [Mate]: independent_wheel_pair:1 ↔ tuleja_M6_M10_7:3
- [Mate]: glowny_wahacz_zewn:2 ↔ independent_wheel_pair:1
- [Mate]: glowny_wahacz_zewn:2 ↔ independent_wheel_pair:1
- [Mate]: glowny_wahacz_zewn:2 ↔ tuleja_M6_M10_7:3
- [Mate]: ramie_1_wahacza:2 ↔ M5_shaft:2
- [Mate]: M6_70_shaft:13 ↔ M6_nut_5mm:61
- [Mate] (5 mm): M6_nut_5mm:60 ↔ M6_nut_5mm:61
- [Mate]: M6_70_shaft:13 ↔ M6_nut_5mm:62
- [Mate] (5 mm): M6_nut_5mm:59 ↔ M6_nut_5mm:62
- [Mate]: M6_70_shaft:14 ↔ M6_nut_5mm:63
- [Mate] (5 mm): M6_nut_5mm:57 ↔ M6_nut_5mm:63
- [Mate]: M6_70_shaft:14 ↔ M6_nut_5mm:64
- [Mate] (5 mm): M6_nut_5mm:58 ↔ M6_nut_5mm:64
- [Mate]: M6_70_shaft:14 ↔ tuleja_M6_M10_6:1
- [Mate]: tuleja_M6_M10_6:1 ↔ M6_nut_5mm:63
- [Mate]: M6_70_shaft:13 ↔ tuleja_M6_M10_6:2
- [Mate]: tuleja_TUF106040:50 ↔ tuleja_M6_M10_6:2
- [Mate]: M6_70_shaft:13 ↔ tuleja_M6_M10_6:3
- [Mate]: tuleja_TUF106040:44 ↔ tuleja_M6_M10_6:3
- [Mate]: M6_70_shaft:14 ↔ tuleja_M6_M10_6:4
- [Mate]: tuleja_TUF106040:47 ↔ tuleja_M6_M10_6:4
- [Mate]: M5_70_shaft:7 ↔ M5_nut_5mm:46
- [Mate] (5 mm): M5_nut_5mm:40 ↔ M5_nut_5mm:46
- [Mate]: M5_70_shaft:7 ↔ M5_nut_5mm:47
- [Mate] (5 mm): M5_nut_5mm:41 ↔ M5_nut_5mm:47
- [Mate]: M5_70_shaft:7 ↔ tuleja_M5_M9_17.5:2
- [Mate]: M5_nut_5mm:47 ↔ tuleja_M5_M9_17.5:2
- [Mate]: M5_70_shaft:7 ↔ tuleja_M5_M9_17.5:1
- [Mate]: Korpus:7 ↔ tuleja_M5_M9_17.5:1
- Zestawiające:1222 [Mate]: plyta_boczna:2 ↔ M6_70_shaft:14
- Zestawiające:1223 [Mate]: glowny_wahacz_zewn:1 ↔ tuleja_M6_M10_7:3
- Zestawiające:1224 [Mate]: plyta_boczna:2 ↔ M6_nut_5mm:58
- Zestawiające:1225 [Mate]: plyta_boczna:2 ↔ M6_70_shaft:13
- Zestawiające:1226 [Mate]: plyta_boczna:2 ↔ tuleja_M5_M9_17.5:2
- Kątowe:27 [Angle] (90 deg): ramie_1_wahacza:2 ↔ glowny_wahacz_zewn:1
- [Mate]: ramie_2_wahacza:3 ↔ tuleja_TUF106040:51
- [Mate]: ramie_2_wahacza:3 ↔ tuleja_TUF106040:51
- [Angle] (0 deg): ramie_2_wahacza:3 ↔ tuleja_TUF106040:51
- [Mate]: ramie_1_wahacza:3 ↔ tuleja_TUF106040:54
- [Mate]: ramie_1_wahacza:3 ↔ tuleja_TUF106040:54
- [Angle] (0 deg): ramie_1_wahacza:3 ↔ tuleja_TUF106040:54
- [Mate]: ramie_2_wahacza:4 ↔ tuleja_TUF106040:57
- [Mate]: ramie_2_wahacza:4 ↔ tuleja_TUF106040:57
- [Angle] (0 deg): ramie_2_wahacza:4 ↔ tuleja_TUF106040:57
- [Mate]: Korpus:8 ↔ Tlok:8
- [Angle] (0 deg): Korpus:8 ↔ Tlok:8
- [Mate]: Korpus:8 ↔ Nakretka:8
- [Mate] (5 mm): Korpus:8 ↔ Nakretka:8
- [CylindricalJoint]: Korpus:8 ↔ Tlok:8
- [Mate]: Korpus:8 ↔ M5_70_shaft:8
- [Flush] (-32.5 mm): Korpus:8 ↔ M5_70_shaft:8
- [Mate]: M5_nut_5mm:48 ↔ M5_70_shaft:8
- [Mate]: M5_70_shaft:8 ↔ M5_nut_5mm:49
- [Mate] (60 mm): M5_nut_5mm:48 ↔ M5_nut_5mm:49
- [Mate] (27.5 mm): Korpus:8 ↔ M5_nut_5mm:48
- [Mate]: tuleja_TUF106040:56 ↔ ramie_1_wahacza:4
- [Mate]: tuleja_TUF106040:55 ↔ ramie_1_wahacza:4
- [Mate]: tuleja_TUF106040:56 ↔ ramie_1_wahacza:4
- [Mate]: tuleja_TUF106040:51 ↔ tuleja_TUF106040:57
- [Mate]: wspornik_amortyzatora:15 ↔ wspornik_amortyzatora:16
- [Mate]: wspornik_amortyzatora:15 ↔ wspornik_amortyzatora:16
- [Mate] (5 mm): wspornik_amortyzatora:15 ↔ wspornik_amortyzatora:16
- [Mate]: M3_16_shaft:8 ↔ wspornik_amortyzatora:16
- [Flush] (-2.5 mm): M3_16_shaft:8 ↔ wspornik_amortyzatora:15
- [Mate]: M3_16_shaft:8 ↔ M3_nut_2,5mm:15
- [Mate]: M3_nut_2,5mm:15 ↔ wspornik_amortyzatora:15
- [Mate]: M3_16_shaft:8 ↔ M3_nut_2,5mm:16
- [Mate]: M3_nut_2,5mm:16 ↔ wspornik_amortyzatora:16
- [Mate]: Tlok:8 ↔ M3_16_shaft:8
- [Mate]: Tlok:8 ↔ wspornik_amortyzatora:16
- [Mate]: ramie_1_wahacza:3 ↔ wspornik_amortyzatora:15
- [Mate]: ramie_1_wahacza:3 ↔ wspornik_amortyzatora:15
- [Mate] (4.5 mm): ramie_1_wahacza:3 ↔ wspornik_amortyzatora:15
- [Mate]: tuleja_TUF106040:54 ↔ M6_40_shaft:3
- [Flush] (7 mm): ramie_1_wahacza:3 ↔ M6_40_shaft:3
- [Mate]: tuleja_TUF106040:57 ↔ M6_40_shaft:4
- [Flush] (7 mm): ramie_2_wahacza:4 ↔ M6_40_shaft:4
- [Mate]: M6_nut_5mm:65 ↔ M6_40_shaft:3
- [Mate]: ramie_1_wahacza:3 ↔ M6_nut_5mm:65
- [Mate]: M6_40_shaft:3 ↔ M6_nut_5mm:66
- [Mate]: ramie_1_wahacza:4 ↔ M6_nut_5mm:66
- [Mate]: M6_40_shaft:4 ↔ M6_nut_5mm:67
- [Mate]: ramie_2_wahacza:3 ↔ M6_nut_5mm:67
- [Mate]: M6_40_shaft:4 ↔ M6_nut_5mm:68
- [Mate]: ramie_2_wahacza:4 ↔ M6_nut_5mm:68
- [Mate]: M6_40_shaft:3 ↔ tuleja_M6_M10_7:4
- [Mate]: M6_40_shaft:4 ↔ tuleja_M6_M10_7:5
- [Mate]: M6_1,25_pad:9 ↔ M6_1,25_pad:10
- [Mate]: M6_1,25_pad:9 ↔ M6_1,25_pad:10
- [Mate]: M6_40_shaft:3 ↔ M6_1,25_pad:9
- [Mate]: M6_1,25_pad:11 ↔ M6_1,25_pad:12
- [Mate]: M6_1,25_pad:11 ↔ M6_1,25_pad:12
- [Mate]: M6_40_shaft:3 ↔ M6_1,25_pad:11
- [Mate]: tuleja_TUF106040:54 ↔ M6_1,25_pad:11
- [Mate]: M6_1,25_pad:13 ↔ M6_1,25_pad:14
- [Mate]: M6_1,25_pad:13 ↔ M6_1,25_pad:14
- [Mate]: M6_40_shaft:4 ↔ M6_1,25_pad:13
- [Mate]: M6_1,25_pad:15 ↔ M6_1,25_pad:16
- [Mate]: M6_1,25_pad:15 ↔ M6_1,25_pad:16
- [Mate]: M6_40_shaft:4 ↔ M6_1,25_pad:15
- [Mate]: tuleja_TUF106040:57 ↔ M6_1,25_pad:15
- [Mate]: M5_70_shaft:8 ↔ M6_70_shaft:15
- [Flush]: M5_70_shaft:8 ↔ M6_70_shaft:16
- [Mate]: M6_70_shaft:16 ↔ M6_nut_5mm:69
- [Mate]: M6_70_shaft:16 ↔ M6_nut_5mm:70
- [Mate] (60 mm): M6_nut_5mm:69 ↔ M6_nut_5mm:70
- [Flush]: M5_nut_5mm:48 ↔ M6_nut_5mm:70
- [Mate] (60 mm): M6_nut_5mm:71 ↔ M6_nut_5mm:72
- [Mate]: M6_nut_5mm:71 ↔ M6_nut_5mm:72
- [Mate]: M6_70_shaft:15 ↔ M6_nut_5mm:71
- [Flush]: M5_nut_5mm:48 ↔ M6_nut_5mm:72
- [Mate]: ramie_1_wahacza:3 ↔ M5_shaft:3
- [Flush] (7 mm): ramie_1_wahacza:3 ↔ M5_shaft:3
- [Mate]: ramie_1_wahacza:3 ↔ M5_shaft:4
- [Flush] (7 mm): ramie_1_wahacza:3 ↔ M5_shaft:4
- [Mate]: M5_shaft:4 ↔ M5_nut_5mm:50
- [Mate]: ramie_1_wahacza:3 ↔ M5_nut_5mm:50
- [Mate]: M5_shaft:3 ↔ M5_nut_5mm:51
- [Mate]: ramie_1_wahacza:3 ↔ M5_nut_5mm:51
- [Mate]: M5_shaft:3 ↔ M5_nut_5mm:52
- [Mate]: ramie_1_wahacza:4 ↔ M5_nut_5mm:52
- [Mate]: M5_shaft:4 ↔ M5_nut_5mm:53
- [Mate]: ramie_1_wahacza:4 ↔ M5_nut_5mm:53
- [Mate]: M5_shaft:3 ↔ tuleja_M5_M9_4,5:5
- [Mate]: ramie_1_wahacza:4 ↔ tuleja_M5_M9_4,5:5
- [Mate]: M5_shaft:3 ↔ tuleja_M5_M9_4,5:6
- [Mate]: ramie_1_wahacza:3 ↔ tuleja_M5_M9_4,5:6
- [Mate]: M5_shaft:4 ↔ tuleja_M5_M9_4,5:7
- [Mate]: ramie_1_wahacza:4 ↔ tuleja_M5_M9_4,5:7
- [Mate]: M5_shaft:4 ↔ tuleja_M5_M9_4,5:8
- [Mate]: ramie_1_wahacza:3 ↔ tuleja_M5_M9_4,5:8
- [Mate]: M6_40_shaft:4 ↔ glowny_wahacz_zewn:3
- [Mate]: tuleja_M6_M10_7:5 ↔ glowny_wahacz_zewn:3
- [Mate]: M6_40_shaft:3 ↔ glowny_wahacz_zewn:3
- [Mate]: M6_40_shaft:4 ↔ glowny_wahacz_zewn:4
- [Mate]: M6_40_shaft:3 ↔ glowny_wahacz_zewn:4
- [Mate]: tuleja_TUF106040:56 ↔ M6_40_shaft:3
- [Mate]: M6_1,25_pad:12 ↔ glowny_wahacz_zewn:4
- [Mate]: M6_1,25_pad:16 ↔ glowny_wahacz_zewn:4
- [Mate]: tuleja_M6_M10_7:4 ↔ glowny_wahacz_zewn:3
- [Mate]: M6_1,25_pad:9 ↔ glowny_wahacz_zewn:3
- [Mate]: tuleja_TUF106040:56 ↔ M6_1,25_pad:10
- [Mate]: M6_1,25_pad:13 ↔ glowny_wahacz_zewn:3
- [Mate]: tuleja_TUF106040:51 ↔ M6_1,25_pad:14
- [Mate]: tuleja_TUF106040:55 ↔ ramie_1_wahacza:4
- [Mate]: tuleja_TUF106040:53 ↔ M6_70_shaft:16
- [Mate]: ramie_1_wahacza:3 ↔ tuleja_TUF106040:53
- [Mate]: ramie_1_wahacza:3 ↔ tuleja_TUF106040:53
- [Mate]: tuleja_TUF106040:52 ↔ M6_70_shaft:15
- [Mate]: ramie_2_wahacza:3 ↔ tuleja_TUF106040:52
- [Mate]: ramie_2_wahacza:3 ↔ tuleja_TUF106040:52
- [Mate]: tuleja_TUF106040:58 ↔ M6_70_shaft:15
- [Mate]: ramie_2_wahacza:4 ↔ tuleja_TUF106040:58
- [Mate]: ramie_2_wahacza:4 ↔ tuleja_TUF106040:58
- [Mate]: ramie_1_wahacza:4 ↔ M5_shaft:4
- [Mate]: M6_70_shaft:15 ↔ M6_nut_5mm:73
- [Mate] (5 mm): M6_nut_5mm:72 ↔ M6_nut_5mm:73
- [Mate]: M6_70_shaft:15 ↔ M6_nut_5mm:74
- [Mate] (5 mm): M6_nut_5mm:71 ↔ M6_nut_5mm:74
- [Mate]: M6_70_shaft:16 ↔ M6_nut_5mm:75
- [Mate] (5 mm): M6_nut_5mm:69 ↔ M6_nut_5mm:75
- [Mate]: M6_70_shaft:16 ↔ M6_nut_5mm:76
- [Mate] (5 mm): M6_nut_5mm:70 ↔ M6_nut_5mm:76
- [Mate]: M6_70_shaft:16 ↔ tuleja_M6_M10_6:5
- [Mate]: tuleja_M6_M10_6:5 ↔ M6_nut_5mm:75
- [Mate]: M6_70_shaft:15 ↔ tuleja_M6_M10_6:6
- [Mate]: tuleja_TUF106040:58 ↔ tuleja_M6_M10_6:6
- [Mate]: M6_70_shaft:15 ↔ tuleja_M6_M10_6:7
- [Mate]: tuleja_TUF106040:52 ↔ tuleja_M6_M10_6:7
- [Mate]: M6_70_shaft:16 ↔ tuleja_M6_M10_6:8
- [Mate]: tuleja_TUF106040:55 ↔ tuleja_M6_M10_6:8
- [Mate]: M5_70_shaft:8 ↔ M5_nut_5mm:54
- [Mate] (5 mm): M5_nut_5mm:48 ↔ M5_nut_5mm:54
- [Mate]: M5_70_shaft:8 ↔ M5_nut_5mm:55
- [Mate] (5 mm): M5_nut_5mm:49 ↔ M5_nut_5mm:55
- [Mate]: M5_70_shaft:8 ↔ tuleja_M5_M9_17.5:4
- [Mate]: M5_nut_5mm:55 ↔ tuleja_M5_M9_17.5:4
- [Mate]: M5_70_shaft:8 ↔ tuleja_M5_M9_17.5:3
- [Mate]: Korpus:8 ↔ tuleja_M5_M9_17.5:3
- [Mate]: ramie_2_wahacza:7 ↔ tuleja_TUF106040:67
- [Mate]: ramie_2_wahacza:7 ↔ tuleja_TUF106040:67
- [Angle] (0 deg): ramie_2_wahacza:7 ↔ tuleja_TUF106040:67
- [Mate]: ramie_1_wahacza:7 ↔ tuleja_TUF106040:70
- [Mate]: ramie_1_wahacza:7 ↔ tuleja_TUF106040:70
- [Angle] (0 deg): ramie_1_wahacza:7 ↔ tuleja_TUF106040:70
- [Mate]: ramie_2_wahacza:8 ↔ tuleja_TUF106040:73
- [Mate]: ramie_2_wahacza:8 ↔ tuleja_TUF106040:73
- [Angle] (0 deg): ramie_2_wahacza:8 ↔ tuleja_TUF106040:73
- [Mate]: Korpus:10 ↔ Tlok:10
- [Angle] (0 deg): Korpus:10 ↔ Tlok:10
- [Mate]: Korpus:10 ↔ Nakretka:10
- [Mate] (5 mm): Korpus:10 ↔ Nakretka:10
- [CylindricalJoint]: Korpus:10 ↔ Tlok:10
- [Mate]: Korpus:10 ↔ M5_70_shaft:10
- [Flush] (-32.5 mm): Korpus:10 ↔ M5_70_shaft:10
- [Mate]: M5_nut_5mm:64 ↔ M5_70_shaft:10
- [Mate]: M5_70_shaft:10 ↔ M5_nut_5mm:65
- [Mate] (60 mm): M5_nut_5mm:64 ↔ M5_nut_5mm:65
- [Mate] (27.5 mm): Korpus:10 ↔ M5_nut_5mm:64
- [Mate]: tuleja_TUF106040:72 ↔ ramie_1_wahacza:8
- [Mate]: tuleja_TUF106040:71 ↔ ramie_1_wahacza:8
- [Mate]: tuleja_TUF106040:72 ↔ ramie_1_wahacza:8
- [Mate]: tuleja_TUF106040:67 ↔ tuleja_TUF106040:73
- [Mate]: wspornik_amortyzatora:19 ↔ wspornik_amortyzatora:20
- [Mate]: wspornik_amortyzatora:19 ↔ wspornik_amortyzatora:20
- [Mate] (5 mm): wspornik_amortyzatora:19 ↔ wspornik_amortyzatora:20
- [Mate]: M3_16_shaft:10 ↔ wspornik_amortyzatora:20
- [Flush] (-2.5 mm): M3_16_shaft:10 ↔ wspornik_amortyzatora:19
- [Mate]: M3_16_shaft:10 ↔ M3_nut_2,5mm:19
- [Mate]: M3_nut_2,5mm:19 ↔ wspornik_amortyzatora:19
- [Mate]: M3_16_shaft:10 ↔ M3_nut_2,5mm:20
- [Mate]: M3_nut_2,5mm:20 ↔ wspornik_amortyzatora:20
- [Mate]: Tlok:10 ↔ M3_16_shaft:10
- [Mate]: Tlok:10 ↔ wspornik_amortyzatora:20
- [Mate]: ramie_1_wahacza:7 ↔ wspornik_amortyzatora:19
- [Mate]: ramie_1_wahacza:7 ↔ wspornik_amortyzatora:19
- [Mate] (4.5 mm): ramie_1_wahacza:7 ↔ wspornik_amortyzatora:19